# Autodesk Inventor assembly: Pen_Mount
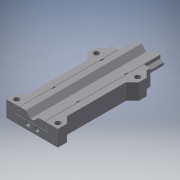
[picture p0: Inventor's stored thumbnail of the model, 180x180]
Saved by Autodesk Inventor 2019 (Build 230136000, 136)
## iProperties
Created: 2021-01-19
Part Number: Pen_Mount
Document SubType Name: Assembly
Designer: zhanb
Author: zhanb
## Documents named in this file (5)
- F:\3D Objects\Inventor\Coursework\ECE HyperRail\Pen_Holder_Assem.iam
- F:\3D Objects\Inventor\Coursework\ECE HyperRail\Holder_Mount.ipt
- F:\3D Objects\Inventor\Coursework\ECE HyperRail\Holder_Slide.ipt
- F:\3D Objects\Inventor\Coursework\ECE HyperRail\Holder_Slide_Top.ipt
- F:\3D Objects\Inventor\Coursework\ECE HyperRail\Pen_Sharpie.ipt
## Components (4 placed, 4 different names)
1. Holder_Mount:1 — Mate:1, Flush:1, Mate:3, Flush:2, Slider:1
2. Holder_Slide:1 — Mate:3, Slider:1, Mate:4, Mate:5, Mate:6, Mate:7, Mate:8
3. Holder_Slide_Top:1 — Mate:4, Mate:5, Mate:8, Mate:9
4. Pen_Sharpie:1 — Mate:6, Mate:7, Mate:9
## Relationships (11: Mate 8, Flush 2, TranslationJoint 1)
- Mate:1: Holder_Mount:1
- Flush:1: Holder_Mount:1
- Mate:3: Holder_Mount:1 ↔ Holder_Slide:1
- Flush:2: Holder_Mount:1
- Slider:1 [TranslationJoint] (0.3175 mm): Holder_Mount:1 ↔ Holder_Slide:1
- Mate:4: Holder_Slide:1 ↔ Holder_Slide_Top:1
- Mate:5 (19.05 mm): Holder_Slide:1 ↔ Holder_Slide_Top:1
- Mate:6 (6.35 mm): Holder_Slide:1 ↔ Pen_Sharpie:1
- Mate:7: Holder_Slide:1 ↔ Pen_Sharpie:1
- Mate:8 (4.572 mm): Holder_Slide:1 ↔ Holder_Slide_Top:1
- Mate:9: Holder_Slide_Top:1 ↔ Pen_Sharpie:1
